(part 1 of 2)
# Autodesk Inventor assembly: Voltage_Regulator_for_ZX60-14LN-S+
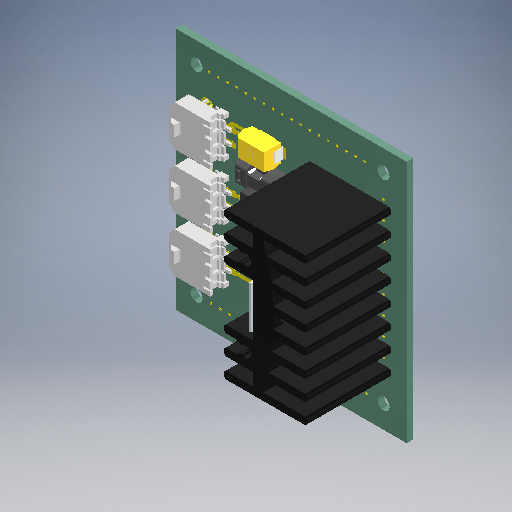
[picture p0: Inventor's stored thumbnail of the model, 512x512]
Saved by Autodesk Inventor 2025.2 (Build 292293000, 293)
## iProperties
Company: Kicad
Created: 2024-11-25
Part Number: Voltage_Regulator_for_ZX60-14LN-S+
Description: KiCad electronic assembly
Document SubType Name: Assembly
Designer: Paul Linke
Authority: Unknown
Sending System: KiCad to STEP converter
Preprocessor: Open CASCADE STEP processor 7.8
Title: Voltage_Regulator_for_ZX60-14LN-S+.step
Author: Pcbnew
## Documents named in this file (257)
- C:\Users\PaulLinke\Documents\Inventor\MyLibrary\Parts\RF-Parts\Voltage_Regulator_for_ZX60-14LN-S+\Voltage_Regulator_for_ZX60-14LN-S+\Voltage_Regulator_for_ZX60-14LN-S+.iam
- C:\Users\PaulLinke\Documents\Inventor\MyLibrary\Parts\RF-Parts\Voltage_Regulator_for_ZX60-14LN-S+\Voltage_Regulator_for_ZX60-14LN-S+\S1M.iam
- C:\Users\PaulLinke\Documents\Inventor\MyLibrary\Parts\RF-Parts\Voltage_Regulator_for_ZX60-14LN-S+\Voltage_Regulator_for_ZX60-14LN-S+\GRM21AR72A334KAC5L.iam
- C:\Users\PaulLinke\Documents\Inventor\MyLibrary\Parts\RF-Parts\Voltage_Regulator_for_ZX60-14LN-S+\Voltage_Regulator_for_ZX60-14LN-S+\43650-0211.iam
- C:\Users\PaulLinke\Documents\Inventor\MyLibrary\Parts\RF-Parts\Voltage_Regulator_for_ZX60-14LN-S+\Voltage_Regulator_for_ZX60-14LN-S+\BA17806CP-E2.iam
- C:\Users\PaulLinke\Documents\Inventor\MyLibrary\Parts\RF-Parts\Voltage_Regulator_for_ZX60-14LN-S+\Voltage_Regulator_for_ZX60-14LN-S+\T491X107K025AT.iam
- C:\Users\PaulLinke\Documents\Inventor\MyLibrary\Parts\RF-Parts\Voltage_Regulator_for_ZX60-14LN-S+\Voltage_Regulator_for_ZX60-14LN-S+\0154001.DRT.iam
- C:\Users\PaulLinke\Documents\Inventor\MyLibrary\Parts\RF-Parts\Voltage_Regulator_for_ZX60-14LN-S+\Voltage_Regulator_for_ZX60-14LN-S+\R_0805_2012Metric.iam
- C:\Users\PaulLinke\Documents\Inventor\MyLibrary\Parts\RF-Parts\Voltage_Regulator_for_ZX60-14LN-S+\Voltage_Regulator_for_ZX60-14LN-S+\GCM21BR72A104KA37L.iam
- C:\Users\PaulLinke\Documents\Inventor\MyLibrary\Parts\RF-Parts\Voltage_Regulator_for_ZX60-14LN-S+\Voltage_Regulator_for_ZX60-14LN-S+\Heatsink_RSPRO-263-251.iam
- C:\Users\PaulLinke\Documents\Inventor\MyLibrary\Parts\RF-Parts\Voltage_Regulator_for_ZX60-14LN-S+\Voltage_Regulator_for_ZX60-14LN-S+\Voltage_Regulator_for_ZX60-14LN-S+_track_1.ipt
- C:\Users\PaulLinke\Documents\Inventor\MyLibrary\Parts\RF-Parts\Voltage_Regulator_for_ZX60-14LN-S+\Voltage_Regulator_for_ZX60-14LN-S+\Voltage_Regulator_for_ZX60-14LN-S+_track_2.ipt
- C:\Users\PaulLinke\Documents\Inventor\MyLibrary\Parts\RF-Parts\Voltage_Regulator_for_ZX60-14LN-S+\Voltage_Regulator_for_ZX60-14LN-S+\Voltage_Regulator_for_ZX60-14LN-S+_track_3.ipt
- C:\Users\PaulLinke\Documents\Inventor\MyLibrary\Parts\RF-Parts\Voltage_Regulator_for_ZX60-14LN-S+\Voltage_Regulator_for_ZX60-14LN-S+\Voltage_Regulator_for_ZX60-14LN-S+_track_4.ipt
- C:\Users\PaulLinke\Documents\Inventor\MyLibrary\Parts\RF-Parts\Voltage_Regulator_for_ZX60-14LN-S+\Voltage_Regulator_for_ZX60-14LN-S+\Voltage_Regulator_for_ZX60-14LN-S+_track_5.ipt
- C:\Users\PaulLinke\Documents\Inventor\MyLibrary\Parts\RF-Parts\Voltage_Regulator_for_ZX60-14LN-S+\Voltage_Regulator_for_ZX60-14LN-S+\Voltage_Regulator_for_ZX60-14LN-S+_track_6.ipt
- C:\Users\PaulLinke\Documents\Inventor\MyLibrary\Parts\RF-Parts\Voltage_Regulator_for_ZX60-14LN-S+\Voltage_Regulator_for_ZX60-14LN-S+\Voltage_Regulator_for_ZX60-14LN-S+_track_7.ipt
- C:\Users\PaulLinke\Documents\Inventor\MyLibrary\Parts\RF-Parts\Voltage_Regulator_for_ZX60-14LN-S+\Voltage_Regulator_for_ZX60-14LN-S+\Voltage_Regulator_for_ZX60-14LN-S+_track_8.ipt
- C:\Users\PaulLinke\Documents\Inventor\MyLibrary\Parts\RF-Parts\Voltage_Regulator_for_ZX60-14LN-S+\Voltage_Regulator_for_ZX60-14LN-S+\Voltage_Regulator_for_ZX60-14LN-S+_track_10.ipt
- C:\Users\PaulLinke\Documents\Inventor\MyLibrary\Parts\RF-Parts\Voltage_Regulator_for_ZX60-14LN-S+\Voltage_Regulator_for_ZX60-14LN-S+\Voltage_Regulator_for_ZX60-14LN-S+_track_11.ipt
- C:\Users\PaulLinke\Documents\Inventor\MyLibrary\Parts\RF-Parts\Voltage_Regulator_for_ZX60-14LN-S+\Voltage_Regulator_for_ZX60-14LN-S+\Voltage_Regulator_for_ZX60-14LN-S+_track_12.ipt
- C:\Users\PaulLinke\Documents\Inventor\MyLibrary\Parts\RF-Parts\Voltage_Regulator_for_ZX60-14LN-S+\Voltage_Regulator_for_ZX60-14LN-S+\Voltage_Regulator_for_ZX60-14LN-S+_track_13.ipt
- C:\Users\PaulLinke\Documents\Inventor\MyLibrary\Parts\RF-Parts\Voltage_Regulator_for_ZX60-14LN-S+\Voltage_Regulator_for_ZX60-14LN-S+\Voltage_Regulator_for_ZX60-14LN-S+_track_14.ipt
- C:\Users\PaulLinke\Documents\Inventor\MyLibrary\Parts\RF-Parts\Voltage_Regulator_for_ZX60-14LN-S+\Voltage_Regulator_for_ZX60-14LN-S+\Voltage_Regulator_for_ZX60-14LN-S+_track_15.ipt
- C:\Users\PaulLinke\Documents\Inventor\MyLibrary\Parts\RF-Parts\Voltage_Regulator_for_ZX60-14LN-S+\Voltage_Regulator_for_ZX60-14LN-S+\Voltage_Regulator_for_ZX60-14LN-S+_track_16.ipt
- C:\Users\PaulLinke\Documents\Inventor\MyLibrary\Parts\RF-Parts\Voltage_Regulator_for_ZX60-14LN-S+\Voltage_Regulator_for_ZX60-14LN-S+\Voltage_Regulator_for_ZX60-14LN-S+_track_17.ipt
- C:\Users\PaulLinke\Documents\Inventor\MyLibrary\Parts\RF-Parts\Voltage_Regulator_for_ZX60-14LN-S+\Voltage_Regulator_for_ZX60-14LN-S+\Voltage_Regulator_for_ZX60-14LN-S+_track_18.ipt
- C:\Users\PaulLinke\Documents\Inventor\MyLibrary\Parts\RF-Parts\Voltage_Regulator_for_ZX60-14LN-S+\Voltage_Regulator_for_ZX60-14LN-S+\Voltage_Regulator_for_ZX60-14LN-S+_track_19.ipt
- C:\Users\PaulLinke\Documents\Inventor\MyLibrary\Parts\RF-Parts\Voltage_Regulator_for_ZX60-14LN-S+\Voltage_Regulator_for_ZX60-14LN-S+\Voltage_Regulator_for_ZX60-14LN-S+_track_20.ipt
- C:\Users\PaulLinke\Documents\Inventor\MyLibrary\Parts\RF-Parts\Voltage_Regulator_for_ZX60-14LN-S+\Voltage_Regulator_for_ZX60-14LN-S+\Voltage_Regulator_for_ZX60-14LN-S+_track_21.ipt
- C:\Users\PaulLinke\Documents\Inventor\MyLibrary\Parts\RF-Parts\Voltage_Regulator_for_ZX60-14LN-S+\Voltage_Regulator_for_ZX60-14LN-S+\Voltage_Regulator_for_ZX60-14LN-S+_track_22.ipt
- C:\Users\PaulLinke\Documents\Inventor\MyLibrary\Parts\RF-Parts\Voltage_Regulator_for_ZX60-14LN-S+\Voltage_Regulator_for_ZX60-14LN-S+\Voltage_Regulator_for_ZX60-14LN-S+_track_23.ipt
- C:\Users\PaulLinke\Documents\Inventor\MyLibrary\Parts\RF-Parts\Voltage_Regulator_for_ZX60-14LN-S+\Voltage_Regulator_for_ZX60-14LN-S+\Voltage_Regulator_for_ZX60-14LN-S+_track_24.ipt
- C:\Users\PaulLinke\Documents\Inventor\MyLibrary\Parts\RF-Parts\Voltage_Regulator_for_ZX60-14LN-S+\Voltage_Regulator_for_ZX60-14LN-S+\Voltage_Regulator_for_ZX60-14LN-S+_track_25.ipt
- C:\Users\PaulLinke\Documents\Inventor\MyLibrary\Parts\RF-Parts\Voltage_Regulator_for_ZX60-14LN-S+\Voltage_Regulator_for_ZX60-14LN-S+\Voltage_Regulator_for_ZX60-14LN-S+_track_27.ipt
- C:\Users\PaulLinke\Documents\Inventor\MyLibrary\Parts\RF-Parts\Voltage_Regulator_for_ZX60-14LN-S+\Voltage_Regulator_for_ZX60-14LN-S+\Voltage_Regulator_for_ZX60-14LN-S+_track_28.ipt
- C:\Users\PaulLinke\Documents\Inventor\MyLibrary\Parts\RF-Parts\Voltage_Regulator_for_ZX60-14LN-S+\Voltage_Regulator_for_ZX60-14LN-S+\Voltage_Regulator_for_ZX60-14LN-S+_track_29.ipt
- C:\Users\PaulLinke\Documents\Inventor\MyLibrary\Parts\RF-Parts\Voltage_Regulator_for_ZX60-14LN-S+\Voltage_Regulator_for_ZX60-14LN-S+\Voltage_Regulator_for_ZX60-14LN-S+_track_30.ipt
- C:\Users\PaulLinke\Documents\Inventor\MyLibrary\Parts\RF-Parts\Voltage_Regulator_for_ZX60-14LN-S+\Voltage_Regulator_for_ZX60-14LN-S+\Voltage_Regulator_for_ZX60-14LN-S+_track_31.ipt
- C:\Users\PaulLinke\Documents\Inventor\MyLibrary\Parts\RF-Parts\Voltage_Regulator_for_ZX60-14LN-S+\Voltage_Regulator_for_ZX60-14LN-S+\Voltage_Regulator_for_ZX60-14LN-S+_track_32.ipt
- C:\Users\PaulLinke\Documents\Inventor\MyLibrary\Parts\RF-Parts\Voltage_Regulator_for_ZX60-14LN-S+\Voltage_Regulator_for_ZX60-14LN-S+\Voltage_Regulator_for_ZX60-14LN-S+_track_33.ipt
- C:\Users\PaulLinke\Documents\Inventor\MyLibrary\Parts\RF-Parts\Voltage_Regulator_for_ZX60-14LN-S+\Voltage_Regulator_for_ZX60-14LN-S+\Voltage_Regulator_for_ZX60-14LN-S+_pad_1.ipt
- C:\Users\PaulLinke\Documents\Inventor\MyLibrary\Parts\RF-Parts\Voltage_Regulator_for_ZX60-14LN-S+\Voltage_Regulator_for_ZX60-14LN-S+\Voltage_Regulator_for_ZX60-14LN-S+_pad_2.ipt
- C:\Users\PaulLinke\Documents\Inventor\MyLibrary\Parts\RF-Parts\Voltage_Regulator_for_ZX60-14LN-S+\Voltage_Regulator_for_ZX60-14LN-S+\Voltage_Regulator_for_ZX60-14LN-S+_pad_3.ipt
- C:\Users\PaulLinke\Documents\Inventor\MyLibrary\Parts\RF-Parts\Voltage_Regulator_for_ZX60-14LN-S+\Voltage_Regulator_for_ZX60-14LN-S+\Voltage_Regulator_for_ZX60-14LN-S+_pad_4.ipt
- C:\Users\PaulLinke\Documents\Inventor\MyLibrary\Parts\RF-Parts\Voltage_Regulator_for_ZX60-14LN-S+\Voltage_Regulator_for_ZX60-14LN-S+\Voltage_Regulator_for_ZX60-14LN-S+_pad_5.ipt
- C:\Users\PaulLinke\Documents\Inventor\MyLibrary\Parts\RF-Parts\Voltage_Regulator_for_ZX60-14LN-S+\Voltage_Regulator_for_ZX60-14LN-S+\Voltage_Regulator_for_ZX60-14LN-S+_pad_6.ipt
- C:\Users\PaulLinke\Documents\Inventor\MyLibrary\Parts\RF-Parts\Voltage_Regulator_for_ZX60-14LN-S+\Voltage_Regulator_for_ZX60-14LN-S+\Voltage_Regulator_for_ZX60-14LN-S+_pad_7.ipt
- C:\Users\PaulLinke\Documents\Inventor\MyLibrary\Parts\RF-Parts\Voltage_Regulator_for_ZX60-14LN-S+\Voltage_Regulator_for_ZX60-14LN-S+\Voltage_Regulator_for_ZX60-14LN-S+_pad_8.ipt
- C:\Users\PaulLinke\Documents\Inventor\MyLibrary\Parts\RF-Parts\Voltage_Regulator_for_ZX60-14LN-S+\Voltage_Regulator_for_ZX60-14LN-S+\Voltage_Regulator_for_ZX60-14LN-S+_pad_9.ipt
- C:\Users\PaulLinke\Documents\Inventor\MyLibrary\Parts\RF-Parts\Voltage_Regulator_for_ZX60-14LN-S+\Voltage_Regulator_for_ZX60-14LN-S+\Voltage_Regulator_for_ZX60-14LN-S+_pad_10.ipt
- C:\Users\PaulLinke\Documents\Inventor\MyLibrary\Parts\RF-Parts\Voltage_Regulator_for_ZX60-14LN-S+\Voltage_Regulator_for_ZX60-14LN-S+\Voltage_Regulator_for_ZX60-14LN-S+_pad_11.ipt
- C:\Users\PaulLinke\Documents\Inventor\MyLibrary\Parts\RF-Parts\Voltage_Regulator_for_ZX60-14LN-S+\Voltage_Regulator_for_ZX60-14LN-S+\Voltage_Regulator_for_ZX60-14LN-S+_pad_12.ipt
- C:\Users\PaulLinke\Documents\Inventor\MyLibrary\Parts\RF-Parts\Voltage_Regulator_for_ZX60-14LN-S+\Voltage_Regulator_for_ZX60-14LN-S+\Voltage_Regulator_for_ZX60-14LN-S+_pad_13.ipt
- C:\Users\PaulLinke\Documents\Inventor\MyLibrary\Parts\RF-Parts\Voltage_Regulator_for_ZX60-14LN-S+\Voltage_Regulator_for_ZX60-14LN-S+\Voltage_Regulator_for_ZX60-14LN-S+_pad_14.ipt
- C:\Users\PaulLinke\Documents\Inventor\MyLibrary\Parts\RF-Parts\Voltage_Regulator_for_ZX60-14LN-S+\Voltage_Regulator_for_ZX60-14LN-S+\Voltage_Regulator_for_ZX60-14LN-S+_pad_15.ipt
- C:\Users\PaulLinke\Documents\Inventor\MyLibrary\Parts\RF-Parts\Voltage_Regulator_for_ZX60-14LN-S+\Voltage_Regulator_for_ZX60-14LN-S+\Voltage_Regulator_for_ZX60-14LN-S+_pad_16.ipt
- C:\Users\PaulLinke\Documents\Inventor\MyLibrary\Parts\RF-Parts\Voltage_Regulator_for_ZX60-14LN-S+\Voltage_Regulator_for_ZX60-14LN-S+\Voltage_Regulator_for_ZX60-14LN-S+_pad_17.ipt
- C:\Users\PaulLinke\Documents\Inventor\MyLibrary\Parts\RF-Parts\Voltage_Regulator_for_ZX60-14LN-S+\Voltage_Regulator_for_ZX60-14LN-S+\Voltage_Regulator_for_ZX60-14LN-S+_pad_18.ipt
- C:\Users\PaulLinke\Documents\Inventor\MyLibrary\Parts\RF-Parts\Voltage_Regulator_for_ZX60-14LN-S+\Voltage_Regulator_for_ZX60-14LN-S+\Voltage_Regulator_for_ZX60-14LN-S+_pad_19.ipt
- C:\Users\PaulLinke\Documents\Inventor\MyLibrary\Parts\RF-Parts\Voltage_Regulator_for_ZX60-14LN-S+\Voltage_Regulator_for_ZX60-14LN-S+\Voltage_Regulator_for_ZX60-14LN-S+_pad_20.ipt
- C:\Users\PaulLinke\Documents\Inventor\MyLibrary\Parts\RF-Parts\Voltage_Regulator_for_ZX60-14LN-S+\Voltage_Regulator_for_ZX60-14LN-S+\Voltage_Regulator_for_ZX60-14LN-S+_pad_21.ipt
- C:\Users\PaulLinke\Documents\Inventor\MyLibrary\Parts\RF-Parts\Voltage_Regulator_for_ZX60-14LN-S+\Voltage_Regulator_for_ZX60-14LN-S+\Voltage_Regulator_for_ZX60-14LN-S+_pad_22.ipt
- C:\Users\PaulLinke\Documents\Inventor\MyLibrary\Parts\RF-Parts\Voltage_Regulator_for_ZX60-14LN-S+\Voltage_Regulator_for_ZX60-14LN-S+\Voltage_Regulator_for_ZX60-14LN-S+_pad_23.ipt
- C:\Users\PaulLinke\Documents\Inventor\MyLibrary\Parts\RF-Parts\Voltage_Regulator_for_ZX60-14LN-S+\Voltage_Regulator_for_ZX60-14LN-S+\Voltage_Regulator_for_ZX60-14LN-S+_pad_24.ipt
- C:\Users\PaulLinke\Documents\Inventor\MyLibrary\Parts\RF-Parts\Voltage_Regulator_for_ZX60-14LN-S+\Voltage_Regulator_for_ZX60-14LN-S+\Voltage_Regulator_for_ZX60-14LN-S+_pad_25.ipt
- C:\Users\PaulLinke\Documents\Inventor\MyLibrary\Parts\RF-Parts\Voltage_Regulator_for_ZX60-14LN-S+\Voltage_Regulator_for_ZX60-14LN-S+\Voltage_Regulator_for_ZX60-14LN-S+_pad_26.ipt
- C:\Users\PaulLinke\Documents\Inventor\MyLibrary\Parts\RF-Parts\Voltage_Regulator_for_ZX60-14LN-S+\Voltage_Regulator_for_ZX60-14LN-S+\Voltage_Regulator_for_ZX60-14LN-S+_pad_27.ipt
- C:\Users\PaulLinke\Documents\Inventor\MyLibrary\Parts\RF-Parts\Voltage_Regulator_for_ZX60-14LN-S+\Voltage_Regulator_for_ZX60-14LN-S+\Voltage_Regulator_for_ZX60-14LN-S+_pad_28.ipt
- C:\Users\PaulLinke\Documents\Inventor\MyLibrary\Parts\RF-Parts\Voltage_Regulator_for_ZX60-14LN-S+\Voltage_Regulator_for_ZX60-14LN-S+\Voltage_Regulator_for_ZX60-14LN-S+_pad_29.ipt
- C:\Users\PaulLinke\Documents\Inventor\MyLibrary\Parts\RF-Parts\Voltage_Regulator_for_ZX60-14LN-S+\Voltage_Regulator_for_ZX60-14LN-S+\Voltage_Regulator_for_ZX60-14LN-S+_pad_30.ipt
- C:\Users\PaulLinke\Documents\Inventor\MyLibrary\Parts\RF-Parts\Voltage_Regulator_for_ZX60-14LN-S+\Voltage_Regulator_for_ZX60-14LN-S+\Voltage_Regulator_for_ZX60-14LN-S+_pad_31.ipt
- C:\Users\PaulLinke\Documents\Inventor\MyLibrary\Parts\RF-Parts\Voltage_Regulator_for_ZX60-14LN-S+\Voltage_Regulator_for_ZX60-14LN-S+\Voltage_Regulator_for_ZX60-14LN-S+_pad_32.ipt
- C:\Users\PaulLinke\Documents\Inventor\MyLibrary\Parts\RF-Parts\Voltage_Regulator_for_ZX60-14LN-S+\Voltage_Regulator_for_ZX60-14LN-S+\Voltage_Regulator_for_ZX60-14LN-S+_pad_33.ipt
- C:\Users\PaulLinke\Documents\Inventor\MyLibrary\Parts\RF-Parts\Voltage_Regulator_for_ZX60-14LN-S+\Voltage_Regulator_for_ZX60-14LN-S+\Voltage_Regulator_for_ZX60-14LN-S+_pad_34.ipt
- C:\Users\PaulLinke\Documents\Inventor\MyLibrary\Parts\RF-Parts\Voltage_Regulator_for_ZX60-14LN-S+\Voltage_Regulator_for_ZX60-14LN-S+\Voltage_Regulator_for_ZX60-14LN-S+_pad_35.ipt
- C:\Users\PaulLinke\Documents\Inventor\MyLibrary\Parts\RF-Parts\Voltage_Regulator_for_ZX60-14LN-S+\Voltage_Regulator_for_ZX60-14LN-S+\Voltage_Regulator_for_ZX60-14LN-S+_pad_36.ipt
- C:\Users\PaulLinke\Documents\Inventor\MyLibrary\Parts\RF-Parts\Voltage_Regulator_for_ZX60-14LN-S+\Voltage_Regulator_for_ZX60-14LN-S+\Voltage_Regulator_for_ZX60-14LN-S+_pad_37.ipt
- C:\Users\PaulLinke\Documents\Inventor\MyLibrary\Parts\RF-Parts\Voltage_Regulator_for_ZX60-14LN-S+\Voltage_Regulator_for_ZX60-14LN-S+\Voltage_Regulator_for_ZX60-14LN-S+_pad_38.ipt
- C:\Users\PaulLinke\Documents\Inventor\MyLibrary\Parts\RF-Parts\Voltage_Regulator_for_ZX60-14LN-S+\Voltage_Regulator_for_ZX60-14LN-S+\Voltage_Regulator_for_ZX60-14LN-S+_pad_39.ipt
- C:\Users\PaulLinke\Documents\Inventor\MyLibrary\Parts\RF-Parts\Voltage_Regulator_for_ZX60-14LN-S+\Voltage_Regulator_for_ZX60-14LN-S+\Voltage_Regulator_for_ZX60-14LN-S+_pad_40.ipt
- C:\Users\PaulLinke\Documents\Inventor\MyLibrary\Parts\RF-Parts\Voltage_Regulator_for_ZX60-14LN-S+\Voltage_Regulator_for_ZX60-14LN-S+\Voltage_Regulator_for_ZX60-14LN-S+_pad_41.ipt
- C:\Users\PaulLinke\Documents\Inventor\MyLibrary\Parts\RF-Parts\Voltage_Regulator_for_ZX60-14LN-S+\Voltage_Regulator_for_ZX60-14LN-S+\Voltage_Regulator_for_ZX60-14LN-S+_pad_42.ipt
- C:\Users\PaulLinke\Documents\Inventor\MyLibrary\Parts\RF-Parts\Voltage_Regulator_for_ZX60-14LN-S+\Voltage_Regulator_for_ZX60-14LN-S+\Voltage_Regulator_for_ZX60-14LN-S+_pad_43.ipt
- C:\Users\PaulLinke\Documents\Inventor\MyLibrary\Parts\RF-Parts\Voltage_Regulator_for_ZX60-14LN-S+\Voltage_Regulator_for_ZX60-14LN-S+\Voltage_Regulator_for_ZX60-14LN-S+_pad_44.ipt
- C:\Users\PaulLinke\Documents\Inventor\MyLibrary\Parts\RF-Parts\Voltage_Regulator_for_ZX60-14LN-S+\Voltage_Regulator_for_ZX60-14LN-S+\Voltage_Regulator_for_ZX60-14LN-S+_pad_45.ipt
- C:\Users\PaulLinke\Documents\Inventor\MyLibrary\Parts\RF-Parts\Voltage_Regulator_for_ZX60-14LN-S+\Voltage_Regulator_for_ZX60-14LN-S+\Voltage_Regulator_for_ZX60-14LN-S+_pad_46.ipt
- C:\Users\PaulLinke\Documents\Inventor\MyLibrary\Parts\RF-Parts\Voltage_Regulator_for_ZX60-14LN-S+\Voltage_Regulator_for_ZX60-14LN-S+\Voltage_Regulator_for_ZX60-14LN-S+_pad_47.ipt
- C:\Users\PaulLinke\Documents\Inventor\MyLibrary\Parts\RF-Parts\Voltage_Regulator_for_ZX60-14LN-S+\Voltage_Regulator_for_ZX60-14LN-S+\Voltage_Regulator_for_ZX60-14LN-S+_pad_48.ipt
- C:\Users\PaulLinke\Documents\Inventor\MyLibrary\Parts\RF-Parts\Voltage_Regulator_for_ZX60-14LN-S+\Voltage_Regulator_for_ZX60-14LN-S+\Voltage_Regulator_for_ZX60-14LN-S+_pad_49.ipt
- C:\Users\PaulLinke\Documents\Inventor\MyLibrary\Parts\RF-Parts\Voltage_Regulator_for_ZX60-14LN-S+\Voltage_Regulator_for_ZX60-14LN-S+\Voltage_Regulator_for_ZX60-14LN-S+_pad_50.ipt
- C:\Users\PaulLinke\Documents\Inventor\MyLibrary\Parts\RF-Parts\Voltage_Regulator_for_ZX60-14LN-S+\Voltage_Regulator_for_ZX60-14LN-S+\Voltage_Regulator_for_ZX60-14LN-S+_pad_51.ipt
- C:\Users\PaulLinke\Documents\Inventor\MyLibrary\Parts\RF-Parts\Voltage_Regulator_for_ZX60-14LN-S+\Voltage_Regulator_for_ZX60-14LN-S+\Voltage_Regulator_for_ZX60-14LN-S+_pad_52.ipt
- C:\Users\PaulLinke\Documents\Inventor\MyLibrary\Parts\RF-Parts\Voltage_Regulator_for_ZX60-14LN-S+\Voltage_Regulator_for_ZX60-14LN-S+\Voltage_Regulator_for_ZX60-14LN-S+_pad_53.ipt
- C:\Users\PaulLinke\Documents\Inventor\MyLibrary\Parts\RF-Parts\Voltage_Regulator_for_ZX60-14LN-S+\Voltage_Regulator_for_ZX60-14LN-S+\Voltage_Regulator_for_ZX60-14LN-S+_pad_54.ipt
- C:\Users\PaulLinke\Documents\Inventor\MyLibrary\Parts\RF-Parts\Voltage_Regulator_for_ZX60-14LN-S+\Voltage_Regulator_for_ZX60-14LN-S+\Voltage_Regulator_for_ZX60-14LN-S+_pad_55.ipt
- C:\Users\PaulLinke\Documents\Inventor\MyLibrary\Parts\RF-Parts\Voltage_Regulator_for_ZX60-14LN-S+\Voltage_Regulator_for_ZX60-14LN-S+\Voltage_Regulator_for_ZX60-14LN-S+_pad_56.ipt
- C:\Users\PaulLinke\Documents\Inventor\MyLibrary\Parts\RF-Parts\Voltage_Regulator_for_ZX60-14LN-S+\Voltage_Regulator_for_ZX60-14LN-S+\Voltage_Regulator_for_ZX60-14LN-S+_pad_57.ipt
- C:\Users\PaulLinke\Documents\Inventor\MyLibrary\Parts\RF-Parts\Voltage_Regulator_for_ZX60-14LN-S+\Voltage_Regulator_for_ZX60-14LN-S+\Voltage_Regulator_for_ZX60-14LN-S+_pad_58.ipt
- C:\Users\PaulLinke\Documents\Inventor\MyLibrary\Parts\RF-Parts\Voltage_Regulator_for_ZX60-14LN-S+\Voltage_Regulator_for_ZX60-14LN-S+\Voltage_Regulator_for_ZX60-14LN-S+_pad_59.ipt
- C:\Users\PaulLinke\Documents\Inventor\MyLibrary\Parts\RF-Parts\Voltage_Regulator_for_ZX60-14LN-S+\Voltage_Regulator_for_ZX60-14LN-S+\Voltage_Regulator_for_ZX60-14LN-S+_pad_60.ipt
- C:\Users\PaulLinke\Documents\Inventor\MyLibrary\Parts\RF-Parts\Voltage_Regulator_for_ZX60-14LN-S+\Voltage_Regulator_for_ZX60-14LN-S+\Voltage_Regulator_for_ZX60-14LN-S+_pad_61.ipt
- C:\Users\PaulLinke\Documents\Inventor\MyLibrary\Parts\RF-Parts\Voltage_Regulator_for_ZX60-14LN-S+\Voltage_Regulator_for_ZX60-14LN-S+\Voltage_Regulator_for_ZX60-14LN-S+_pad_62.ipt
- C:\Users\PaulLinke\Documents\Inventor\MyLibrary\Parts\RF-Parts\Voltage_Regulator_for_ZX60-14LN-S+\Voltage_Regulator_for_ZX60-14LN-S+\Voltage_Regulator_for_ZX60-14LN-S+_pad_63.ipt
- C:\Users\PaulLinke\Documents\Inventor\MyLibrary\Parts\RF-Parts\Voltage_Regulator_for_ZX60-14LN-S+\Voltage_Regulator_for_ZX60-14LN-S+\Voltage_Regulator_for_ZX60-14LN-S+_pad_64.ipt
- C:\Users\PaulLinke\Documents\Inventor\MyLibrary\Parts\RF-Parts\Voltage_Regulator_for_ZX60-14LN-S+\Voltage_Regulator_for_ZX60-14LN-S+\Voltage_Regulator_for_ZX60-14LN-S+_pad_65.ipt
- C:\Users\PaulLinke\Documents\Inventor\MyLibrary\Parts\RF-Parts\Voltage_Regulator_for_ZX60-14LN-S+\Voltage_Regulator_for_ZX60-14LN-S+\Voltage_Regulator_for_ZX60-14LN-S+_pad_66.ipt
- C:\Users\PaulLinke\Documents\Inventor\MyLibrary\Parts\RF-Parts\Voltage_Regulator_for_ZX60-14LN-S+\Voltage_Regulator_for_ZX60-14LN-S+\Voltage_Regulator_for_ZX60-14LN-S+_pad_67.ipt
- C:\Users\PaulLinke\Documents\Inventor\MyLibrary\Parts\RF-Parts\Voltage_Regulator_for_ZX60-14LN-S+\Voltage_Regulator_for_ZX60-14LN-S+\Voltage_Regulator_for_ZX60-14LN-S+_pad_68.ipt
- C:\Users\PaulLinke\Documents\Inventor\MyLibrary\Parts\RF-Parts\Voltage_Regulator_for_ZX60-14LN-S+\Voltage_Regulator_for_ZX60-14LN-S+\Voltage_Regulator_for_ZX60-14LN-S+_pad_69.ipt
- C:\Users\PaulLinke\Documents\Inventor\MyLibrary\Parts\RF-Parts\Voltage_Regulator_for_ZX60-14LN-S+\Voltage_Regulator_for_ZX60-14LN-S+\Voltage_Regulator_for_ZX60-14LN-S+_pad_70.ipt
- C:\Users\PaulLinke\Documents\Inventor\MyLibrary\Parts\RF-Parts\Voltage_Regulator_for_ZX60-14LN-S+\Voltage_Regulator_for_ZX60-14LN-S+\Voltage_Regulator_for_ZX60-14LN-S+_pad_71.ipt
- C:\Users\PaulLinke\Documents\Inventor\MyLibrary\Parts\RF-Parts\Voltage_Regulator_for_ZX60-14LN-S+\Voltage_Regulator_for_ZX60-14LN-S+\Voltage_Regulator_for_ZX60-14LN-S+_pad_72.ipt
- C:\Users\PaulLinke\Documents\Inventor\MyLibrary\Parts\RF-Parts\Voltage_Regulator_for_ZX60-14LN-S+\Voltage_Regulator_for_ZX60-14LN-S+\Voltage_Regulator_for_ZX60-14LN-S+_pad_73.ipt
- C:\Users\PaulLinke\Documents\Inventor\MyLibrary\Parts\RF-Parts\Voltage_Regulator_for_ZX60-14LN-S+\Voltage_Regulator_for_ZX60-14LN-S+\Voltage_Regulator_for_ZX60-14LN-S+_pad_74.ipt
- C:\Users\PaulLinke\Documents\Inventor\MyLibrary\Parts\RF-Parts\Voltage_Regulator_for_ZX60-14LN-S+\Voltage_Regulator_for_ZX60-14LN-S+\Voltage_Regulator_for_ZX60-14LN-S+_pad_75.ipt
- C:\Users\PaulLinke\Documents\Inventor\MyLibrary\Parts\RF-Parts\Voltage_Regulator_for_ZX60-14LN-S+\Voltage_Regulator_for_ZX60-14LN-S+\Voltage_Regulator_for_ZX60-14LN-S+_pad_76.ipt
- C:\Users\PaulLinke\Documents\Inventor\MyLibrary\Parts\RF-Parts\Voltage_Regulator_for_ZX60-14LN-S+\Voltage_Regulator_for_ZX60-14LN-S+\Voltage_Regulator_for_ZX60-14LN-S+_pad_77.ipt
- C:\Users\PaulLinke\Documents\Inventor\MyLibrary\Parts\RF-Parts\Voltage_Regulator_for_ZX60-14LN-S+\Voltage_Regulator_for_ZX60-14LN-S+\Voltage_Regulator_for_ZX60-14LN-S+_pad_78.ipt
- C:\Users\PaulLinke\Documents\Inventor\MyLibrary\Parts\RF-Parts\Voltage_Regulator_for_ZX60-14LN-S+\Voltage_Regulator_for_ZX60-14LN-S+\Voltage_Regulator_for_ZX60-14LN-S+_pad_79.ipt
- C:\Users\PaulLinke\Documents\Inventor\MyLibrary\Parts\RF-Parts\Voltage_Regulator_for_ZX60-14LN-S+\Voltage_Regulator_for_ZX60-14LN-S+\Voltage_Regulator_for_ZX60-14LN-S+_pad_80.ipt
- C:\Users\PaulLinke\Documents\Inventor\MyLibrary\Parts\RF-Parts\Voltage_Regulator_for_ZX60-14LN-S+\Voltage_Regulator_for_ZX60-14LN-S+\Voltage_Regulator_for_ZX60-14LN-S+_pad_81.ipt
- C:\Users\PaulLinke\Documents\Inventor\MyLibrary\Parts\RF-Parts\Voltage_Regulator_for_ZX60-14LN-S+\Voltage_Regulator_for_ZX60-14LN-S+\Voltage_Regulator_for_ZX60-14LN-S+_pad_82.ipt
- C:\Users\PaulLinke\Documents\Inventor\MyLibrary\Parts\RF-Parts\Voltage_Regulator_for_ZX60-14LN-S+\Voltage_Regulator_for_ZX60-14LN-S+\Voltage_Regulator_for_ZX60-14LN-S+_pad_83.ipt
- C:\Users\PaulLinke\Documents\Inventor\MyLibrary\Parts\RF-Parts\Voltage_Regulator_for_ZX60-14LN-S+\Voltage_Regulator_for_ZX60-14LN-S+\Voltage_Regulator_for_ZX60-14LN-S+_pad_84.ipt
- C:\Users\PaulLinke\Documents\Inventor\MyLibrary\Parts\RF-Parts\Voltage_Regulator_for_ZX60-14LN-S+\Voltage_Regulator_for_ZX60-14LN-S+\Voltage_Regulator_for_ZX60-14LN-S+_pad_85.ipt
- C:\Users\PaulLinke\Documents\Inventor\MyLibrary\Parts\RF-Parts\Voltage_Regulator_for_ZX60-14LN-S+\Voltage_Regulator_for_ZX60-14LN-S+\Voltage_Regulator_for_ZX60-14LN-S+_pad_86.ipt
- C:\Users\PaulLinke\Documents\Inventor\MyLibrary\Parts\RF-Parts\Voltage_Regulator_for_ZX60-14LN-S+\Voltage_Regulator_for_ZX60-14LN-S+\Voltage_Regulator_for_ZX60-14LN-S+_pad_87.ipt
- C:\Users\PaulLinke\Documents\Inventor\MyLibrary\Parts\RF-Parts\Voltage_Regulator_for_ZX60-14LN-S+\Voltage_Regulator_for_ZX60-14LN-S+\Voltage_Regulator_for_ZX60-14LN-S+_pad_88.ipt
- C:\Users\PaulLinke\Documents\Inventor\MyLibrary\Parts\RF-Parts\Voltage_Regulator_for_ZX60-14LN-S+\Voltage_Regulator_for_ZX60-14LN-S+\Voltage_Regulator_for_ZX60-14LN-S+_pad_89.ipt
- C:\Users\PaulLinke\Documents\Inventor\MyLibrary\Parts\RF-Parts\Voltage_Regulator_for_ZX60-14LN-S+\Voltage_Regulator_for_ZX60-14LN-S+\Voltage_Regulator_for_ZX60-14LN-S+_pad_90.ipt
- C:\Users\PaulLinke\Documents\Inventor\MyLibrary\Parts\RF-Parts\Voltage_Regulator_for_ZX60-14LN-S+\Voltage_Regulator_for_ZX60-14LN-S+\Voltage_Regulator_for_ZX60-14LN-S+_pad_91.ipt
- C:\Users\PaulLinke\Documents\Inventor\MyLibrary\Parts\RF-Parts\Voltage_Regulator_for_ZX60-14LN-S+\Voltage_Regulator_for_ZX60-14LN-S+\Voltage_Regulator_for_ZX60-14LN-S+_pad_92.ipt
- C:\Users\PaulLinke\Documents\Inventor\MyLibrary\Parts\RF-Parts\Voltage_Regulator_for_ZX60-14LN-S+\Voltage_Regulator_for_ZX60-14LN-S+\Voltage_Regulator_for_ZX60-14LN-S+_pad_93.ipt
- C:\Users\PaulLinke\Documents\Inventor\MyLibrary\Parts\RF-Parts\Voltage_Regulator_for_ZX60-14LN-S+\Voltage_Regulator_for_ZX60-14LN-S+\Voltage_Regulator_for_ZX60-14LN-S+_pad_94.ipt
- C:\Users\PaulLinke\Documents\Inventor\MyLibrary\Parts\RF-Parts\Voltage_Regulator_for_ZX60-14LN-S+\Voltage_Regulator_for_ZX60-14LN-S+\Voltage_Regulator_for_ZX60-14LN-S+_pad_95.ipt
- C:\Users\PaulLinke\Documents\Inventor\MyLibrary\Parts\RF-Parts\Voltage_Regulator_for_ZX60-14LN-S+\Voltage_Regulator_for_ZX60-14LN-S+\Voltage_Regulator_for_ZX60-14LN-S+_pad_96.ipt
- C:\Users\PaulLinke\Documents\Inventor\MyLibrary\Parts\RF-Parts\Voltage_Regulator_for_ZX60-14LN-S+\Voltage_Regulator_for_ZX60-14LN-S+\Voltage_Regulator_for_ZX60-14LN-S+_pad_97.ipt
- C:\Users\PaulLinke\Documents\Inventor\MyLibrary\Parts\RF-Parts\Voltage_Regulator_for_ZX60-14LN-S+\Voltage_Regulator_for_ZX60-14LN-S+\Voltage_Regulator_for_ZX60-14LN-S+_pad_98.ipt
- C:\Users\PaulLinke\Documents\Inventor\MyLibrary\Parts\RF-Parts\Voltage_Regulator_for_ZX60-14LN-S+\Voltage_Regulator_for_ZX60-14LN-S+\Voltage_Regulator_for_ZX60-14LN-S+_pad_99.ipt
- C:\Users\PaulLinke\Documents\Inventor\MyLibrary\Parts\RF-Parts\Voltage_Regulator_for_ZX60-14LN-S+\Voltage_Regulator_for_ZX60-14LN-S+\Voltage_Regulator_for_ZX60-14LN-S+_pad_100.ipt
- C:\Users\PaulLinke\Documents\Inventor\MyLibrary\Parts\RF-Parts\Voltage_Regulator_for_ZX60-14LN-S+\Voltage_Regulator_for_ZX60-14LN-S+\Voltage_Regulator_for_ZX60-14LN-S+_pad_101.ipt
- C:\Users\PaulLinke\Documents\Inventor\MyLibrary\Parts\RF-Parts\Voltage_Regulator_for_ZX60-14LN-S+\Voltage_Regulator_for_ZX60-14LN-S+\Voltage_Regulator_for_ZX60-14LN-S+_pad_102.ipt
- C:\Users\PaulLinke\Documents\Inventor\MyLibrary\Parts\RF-Parts\Voltage_Regulator_for_ZX60-14LN-S+\Voltage_Regulator_for_ZX60-14LN-S+\Voltage_Regulator_for_ZX60-14LN-S+_pad_103.ipt
- C:\Users\PaulLinke\Documents\Inventor\MyLibrary\Parts\RF-Parts\Voltage_Regulator_for_ZX60-14LN-S+\Voltage_Regulator_for_ZX60-14LN-S+\Voltage_Regulator_for_ZX60-14LN-S+_pad_104.ipt
- C:\Users\PaulLinke\Documents\Inventor\MyLibrary\Parts\RF-Parts\Voltage_Regulator_for_ZX60-14LN-S+\Voltage_Regulator_for_ZX60-14LN-S+\Voltage_Regulator_for_ZX60-14LN-S+_pad_105.ipt
- C:\Users\PaulLinke\Documents\Inventor\MyLibrary\Parts\RF-Parts\Voltage_Regulator_for_ZX60-14LN-S+\Voltage_Regulator_for_ZX60-14LN-S+\Voltage_Regulator_for_ZX60-14LN-S+_pad_106.ipt
- C:\Users\PaulLinke\Documents\Inventor\MyLibrary\Parts\RF-Parts\Voltage_Regulator_for_ZX60-14LN-S+\Voltage_Regulator_for_ZX60-14LN-S+\Voltage_Regulator_for_ZX60-14LN-S+_pad_107.ipt
- C:\Users\PaulLinke\Documents\Inventor\MyLibrary\Parts\RF-Parts\Voltage_Regulator_for_ZX60-14LN-S+\Voltage_Regulator_for_ZX60-14LN-S+\Voltage_Regulator_for_ZX60-14LN-S+_pad_108.ipt
- C:\Users\PaulLinke\Documents\Inventor\MyLibrary\Parts\RF-Parts\Voltage_Regulator_for_ZX60-14LN-S+\Voltage_Regulator_for_ZX60-14LN-S+\Voltage_Regulator_for_ZX60-14LN-S+_pad_109.ipt
- C:\Users\PaulLinke\Documents\Inventor\MyLibrary\Parts\RF-Parts\Voltage_Regulator_for_ZX60-14LN-S+\Voltage_Regulator_for_ZX60-14LN-S+\Voltage_Regulator_for_ZX60-14LN-S+_pad_110.ipt
- C:\Users\PaulLinke\Documents\Inventor\MyLibrary\Parts\RF-Parts\Voltage_Regulator_for_ZX60-14LN-S+\Voltage_Regulator_for_ZX60-14LN-S+\Voltage_Regulator_for_ZX60-14LN-S+_pad_111.ipt
- C:\Users\PaulLinke\Documents\Inventor\MyLibrary\Parts\RF-Parts\Voltage_Regulator_for_ZX60-14LN-S+\Voltage_Regulator_for_ZX60-14LN-S+\Voltage_Regulator_for_ZX60-14LN-S+_pad_112.ipt
- C:\Users\PaulLinke\Documents\Inventor\MyLibrary\Parts\RF-Parts\Voltage_Regulator_for_ZX60-14LN-S+\Voltage_Regulator_for_ZX60-14LN-S+\Voltage_Regulator_for_ZX60-14LN-S+_pad_113.ipt
- C:\Users\PaulLinke\Documents\Inventor\MyLibrary\Parts\RF-Parts\Voltage_Regulator_for_ZX60-14LN-S+\Voltage_Regulator_for_ZX60-14LN-S+\Voltage_Regulator_for_ZX60-14LN-S+_pad_114.ipt
- C:\Users\PaulLinke\Documents\Inventor\MyLibrary\Parts\RF-Parts\Voltage_Regulator_for_ZX60-14LN-S+\Voltage_Regulator_for_ZX60-14LN-S+\Voltage_Regulator_for_ZX60-14LN-S+_pad_115.ipt
- C:\Users\PaulLinke\Documents\Inventor\MyLibrary\Parts\RF-Parts\Voltage_Regulator_for_ZX60-14LN-S+\Voltage_Regulator_for_ZX60-14LN-S+\Voltage_Regulator_for_ZX60-14LN-S+_pad_116.ipt
- C:\Users\PaulLinke\Documents\Inventor\MyLibrary\Parts\RF-Parts\Voltage_Regulator_for_ZX60-14LN-S+\Voltage_Regulator_for_ZX60-14LN-S+\Voltage_Regulator_for_ZX60-14LN-S+_pad_117.ipt
- C:\Users\PaulLinke\Documents\Inventor\MyLibrary\Parts\RF-Parts\Voltage_Regulator_for_ZX60-14LN-S+\Voltage_Regulator_for_ZX60-14LN-S+\Voltage_Regulator_for_ZX60-14LN-S+_pad_118.ipt
- C:\Users\PaulLinke\Documents\Inventor\MyLibrary\Parts\RF-Parts\Voltage_Regulator_for_ZX60-14LN-S+\Voltage_Regulator_for_ZX60-14LN-S+\Voltage_Regulator_for_ZX60-14LN-S+_pad_119.ipt
- C:\Users\PaulLinke\Documents\Inventor\MyLibrary\Parts\RF-Parts\Voltage_Regulator_for_ZX60-14LN-S+\Voltage_Regulator_for_ZX60-14LN-S+\Voltage_Regulator_for_ZX60-14LN-S+_pad_120.ipt
- C:\Users\PaulLinke\Documents\Inventor\MyLibrary\Parts\RF-Parts\Voltage_Regulator_for_ZX60-14LN-S+\Voltage_Regulator_for_ZX60-14LN-S+\Voltage_Regulator_for_ZX60-14LN-S+_pad_121.ipt
- C:\Users\PaulLinke\Documents\Inventor\MyLibrary\Parts\RF-Parts\Voltage_Regulator_for_ZX60-14LN-S+\Voltage_Regulator_for_ZX60-14LN-S+\Voltage_Regulator_for_ZX60-14LN-S+_pad_122.ipt
- C:\Users\PaulLinke\Documents\Inventor\MyLibrary\Parts\RF-Parts\Voltage_Regulator_for_ZX60-14LN-S+\Voltage_Regulator_for_ZX60-14LN-S+\Voltage_Regulator_for_ZX60-14LN-S+_pad_123.ipt
- C:\Users\PaulLinke\Documents\Inventor\MyLibrary\Parts\RF-Parts\Voltage_Regulator_for_ZX60-14LN-S+\Voltage_Regulator_for_ZX60-14LN-S+\Voltage_Regulator_for_ZX60-14LN-S+_pad_124.ipt
- C:\Users\PaulLinke\Documents\Inventor\MyLibrary\Parts\RF-Parts\Voltage_Regulator_for_ZX60-14LN-S+\Voltage_Regulator_for_ZX60-14LN-S+\Voltage_Regulator_for_ZX60-14LN-S+_pad_125.ipt
- C:\Users\PaulLinke\Documents\Inventor\MyLibrary\Parts\RF-Parts\Voltage_Regulator_for_ZX60-14LN-S+\Voltage_Regulator_for_ZX60-14LN-S+\Voltage_Regulator_for_ZX60-14LN-S+_pad_126.ipt
- C:\Users\PaulLinke\Documents\Inventor\MyLibrary\Parts\RF-Parts\Voltage_Regulator_for_ZX60-14LN-S+\Voltage_Regulator_for_ZX60-14LN-S+\Voltage_Regulator_for_ZX60-14LN-S+_pad_127.ipt
- C:\Users\PaulLinke\Documents\Inventor\MyLibrary\Parts\RF-Parts\Voltage_Regulator_for_ZX60-14LN-S+\Voltage_Regulator_for_ZX60-14LN-S+\Voltage_Regulator_for_ZX60-14LN-S+_pad_128.ipt
- C:\Users\PaulLinke\Documents\Inventor\MyLibrary\Parts\RF-Parts\Voltage_Regulator_for_ZX60-14LN-S+\Voltage_Regulator_for_ZX60-14LN-S+\Voltage_Regulator_for_ZX60-14LN-S+_pad_129.ipt
- C:\Users\PaulLinke\Documents\Inventor\MyLibrary\Parts\RF-Parts\Voltage_Regulator_for_ZX60-14LN-S+\Voltage_Regulator_for_ZX60-14LN-S+\Voltage_Regulator_for_ZX60-14LN-S+_pad_130.ipt
- C:\Users\PaulLinke\Documents\Inventor\MyLibrary\Parts\RF-Parts\Voltage_Regulator_for_ZX60-14LN-S+\Voltage_Regulator_for_ZX60-14LN-S+\Voltage_Regulator_for_ZX60-14LN-S+_pad_131.ipt
- C:\Users\PaulLinke\Documents\Inventor\MyLibrary\Parts\RF-Parts\Voltage_Regulator_for_ZX60-14LN-S+\Voltage_Regulator_for_ZX60-14LN-S+\Voltage_Regulator_for_ZX60-14LN-S+_pad_132.ipt
- C:\Users\PaulLinke\Documents\Inventor\MyLibrary\Parts\RF-Parts\Voltage_Regulator_for_ZX60-14LN-S+\Voltage_Regulator_for_ZX60-14LN-S+\Voltage_Regulator_for_ZX60-14LN-S+_pad_133.ipt
- C:\Users\PaulLinke\Documents\Inventor\MyLibrary\Parts\RF-Parts\Voltage_Regulator_for_ZX60-14LN-S+\Voltage_Regulator_for_ZX60-14LN-S+\Voltage_Regulator_for_ZX60-14LN-S+_pad_134.ipt
- C:\Users\PaulLinke\Documents\Inventor\MyLibrary\Parts\RF-Parts\Voltage_Regulator_for_ZX60-14LN-S+\Voltage_Regulator_for_ZX60-14LN-S+\Voltage_Regulator_for_ZX60-14LN-S+_pad_135.ipt
- C:\Users\PaulLinke\Documents\Inventor\MyLibrary\Parts\RF-Parts\Voltage_Regulator_for_ZX60-14LN-S+\Voltage_Regulator_for_ZX60-14LN-S+\Voltage_Regulator_for_ZX60-14LN-S+_pad_136.ipt
- C:\Users\PaulLinke\Documents\Inventor\MyLibrary\Parts\RF-Parts\Voltage_Regulator_for_ZX60-14LN-S+\Voltage_Regulator_for_ZX60-14LN-S+\Voltage_Regulator_for_ZX60-14LN-S+_pad_137.ipt
- C:\Users\PaulLinke\Documents\Inventor\MyLibrary\Parts\RF-Parts\Voltage_Regulator_for_ZX60-14LN-S+\Voltage_Regulator_for_ZX60-14LN-S+\Voltage_Regulator_for_ZX60-14LN-S+_pad_138.ipt
- C:\Users\PaulLinke\Documents\Inventor\MyLibrary\Parts\RF-Parts\Voltage_Regulator_for_ZX60-14LN-S+\Voltage_Regulator_for_ZX60-14LN-S+\Voltage_Regulator_for_ZX60-14LN-S+_pad_139.ipt
- C:\Users\PaulLinke\Documents\Inventor\MyLibrary\Parts\RF-Parts\Voltage_Regulator_for_ZX60-14LN-S+\Voltage_Regulator_for_ZX60-14LN-S+\Voltage_Regulator_for_ZX60-14LN-S+_pad_140.ipt
- C:\Users\PaulLinke\Documents\Inventor\MyLibrary\Parts\RF-Parts\Voltage_Regulator_for_ZX60-14LN-S+\Voltage_Regulator_for_ZX60-14LN-S+\Voltage_Regulator_for_ZX60-14LN-S+_pad_141.ipt
- C:\Users\PaulLinke\Documents\Inventor\MyLibrary\Parts\RF-Parts\Voltage_Regulator_for_ZX60-14LN-S+\Voltage_Regulator_for_ZX60-14LN-S+\Voltage_Regulator_for_ZX60-14LN-S+_pad_142.ipt
- C:\Users\PaulLinke\Documents\Inventor\MyLibrary\Parts\RF-Parts\Voltage_Regulator_for_ZX60-14LN-S+\Voltage_Regulator_for_ZX60-14LN-S+\Voltage_Regulator_for_ZX60-14LN-S+_pad_143.ipt
- C:\Users\PaulLinke\Documents\Inventor\MyLibrary\Parts\RF-Parts\Voltage_Regulator_for_ZX60-14LN-S+\Voltage_Regulator_for_ZX60-14LN-S+\Voltage_Regulator_for_ZX60-14LN-S+_pad_144.ipt
- C:\Users\PaulLinke\Documents\Inventor\MyLibrary\Parts\RF-Parts\Voltage_Regulator_for_ZX60-14LN-S+\Voltage_Regulator_for_ZX60-14LN-S+\Voltage_Regulator_for_ZX60-14LN-S+_pad_145.ipt
- C:\Users\PaulLinke\Documents\Inventor\MyLibrary\Parts\RF-Parts\Voltage_Regulator_for_ZX60-14LN-S+\Voltage_Regulator_for_ZX60-14LN-S+\Voltage_Regulator_for_ZX60-14LN-S+_pad_146.ipt
- C:\Users\PaulLinke\Documents\Inventor\MyLibrary\Parts\RF-Parts\Voltage_Regulator_for_ZX60-14LN-S+\Voltage_Regulator_for_ZX60-14LN-S+\Voltage_Regulator_for_ZX60-14LN-S+_pad_147.ipt
- C:\Users\PaulLinke\Documents\Inventor\MyLibrary\Parts\RF-Parts\Voltage_Regulator_for_ZX60-14LN-S+\Voltage_Regulator_for_ZX60-14LN-S+\Voltage_Regulator_for_ZX60-14LN-S+_pad_148.ipt
- C:\Users\PaulLinke\Documents\Inventor\MyLibrary\Parts\RF-Parts\Voltage_Regulator_for_ZX60-14LN-S+\Voltage_Regulator_for_ZX60-14LN-S+\Voltage_Regulator_for_ZX60-14LN-S+_pad_149.ipt
- C:\Users\PaulLinke\Documents\Inventor\MyLibrary\Parts\RF-Parts\Voltage_Regulator_for_ZX60-14LN-S+\Voltage_Regulator_for_ZX60-14LN-S+\Voltage_Regulator_for_ZX60-14LN-S+_pad_150.ipt
- C:\Users\PaulLinke\Documents\Inventor\MyLibrary\Parts\RF-Parts\Voltage_Regulator_for_ZX60-14LN-S+\Voltage_Regulator_for_ZX60-14LN-S+\Voltage_Regulator_for_ZX60-14LN-S+_pad_151.ipt
- C:\Users\PaulLinke\Documents\Inventor\MyLibrary\Parts\RF-Parts\Voltage_Regulator_for_ZX60-14LN-S+\Voltage_Regulator_for_ZX60-14LN-S+\Voltage_Regulator_for_ZX60-14LN-S+_pad_152.ipt
- C:\Users\PaulLinke\Documents\Inventor\MyLibrary\Parts\RF-Parts\Voltage_Regulator_for_ZX60-14LN-S+\Voltage_Regulator_for_ZX60-14LN-S+\Voltage_Regulator_for_ZX60-14LN-S+_pad_153.ipt
- C:\Users\PaulLinke\Documents\Inventor\MyLibrary\Parts\RF-Parts\Voltage_Regulator_for_ZX60-14LN-S+\Voltage_Regulator_for_ZX60-14LN-S+\Voltage_Regulator_for_ZX60-14LN-S+_pad_154.ipt
- C:\Users\PaulLinke\Documents\Inventor\MyLibrary\Parts\RF-Parts\Voltage_Regulator_for_ZX60-14LN-S+\Voltage_Regulator_for_ZX60-14LN-S+\Voltage_Regulator_for_ZX60-14LN-S+_pad_155.ipt
- C:\Users\PaulLinke\Documents\Inventor\MyLibrary\Parts\RF-Parts\Voltage_Regulator_for_ZX60-14LN-S+\Voltage_Regulator_for_ZX60-14LN-S+\Voltage_Regulator_for_ZX60-14LN-S+_pad_156.ipt
- C:\Users\PaulLinke\Documents\Inventor\MyLibrary\Parts\RF-Parts\Voltage_Regulator_for_ZX60-14LN-S+\Voltage_Regulator_for_ZX60-14LN-S+\Voltage_Regulator_for_ZX60-14LN-S+_pad_157.ipt
- C:\Users\PaulLinke\Documents\Inventor\MyLibrary\Parts\RF-Parts\Voltage_Regulator_for_ZX60-14LN-S+\Voltage_Regulator_for_ZX60-14LN-S+\Voltage_Regulator_for_ZX60-14LN-S+_pad_158.ipt
- C:\Users\PaulLinke\Documents\Inventor\MyLibrary\Parts\RF-Parts\Voltage_Regulator_for_ZX60-14LN-S+\Voltage_Regulator_for_ZX60-14LN-S+\Voltage_Regulator_for_ZX60-14LN-S+_pad_159.ipt
- C:\Users\PaulLinke\Documents\Inventor\MyLibrary\Parts\RF-Parts\Voltage_Regulator_for_ZX60-14LN-S+\Voltage_Regulator_for_ZX60-14LN-S+\Voltage_Regulator_for_ZX60-14LN-S+_pad_160.ipt
- C:\Users\PaulLinke\Documents\Inventor\MyLibrary\Parts\RF-Parts\Voltage_Regulator_for_ZX60-14LN-S+\Voltage_Regulator_for_ZX60-14LN-S+\Voltage_Regulator_for_ZX60-14LN-S+_pad_161.ipt
- C:\Users\PaulLinke\Documents\Inventor\MyLibrary\Parts\RF-Parts\Voltage_Regulator_for_ZX60-14LN-S+\Voltage_Regulator_for_ZX60-14LN-S+\Voltage_Regulator_for_ZX60-14LN-S+_pad_162.ipt
- C:\Users\PaulLinke\Documents\Inventor\MyLibrary\Parts\RF-Parts\Voltage_Regulator_for_ZX60-14LN-S+\Voltage_Regulator_for_ZX60-14LN-S+\Voltage_Regulator_for_ZX60-14LN-S+_pad_163.ipt
- C:\Users\PaulLinke\Documents\Inventor\MyLibrary\Parts\RF-Parts\Voltage_Regulator_for_ZX60-14LN-S+\Voltage_Regulator_for_ZX60-14LN-S+\Voltage_Regulator_for_ZX60-14LN-S+_pad_164.ipt